# Autodesk Inventor assembly: RPI_2
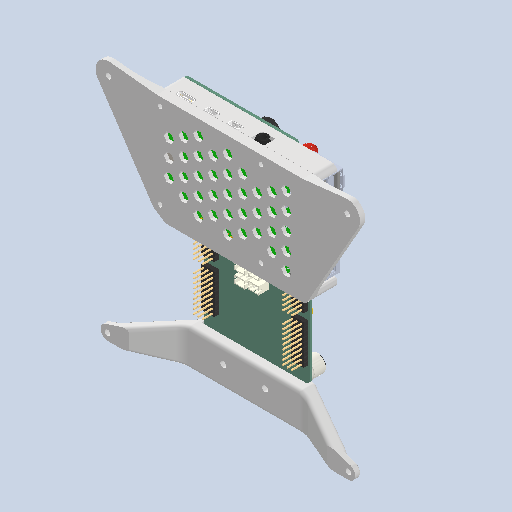
[picture p0: Inventor's stored thumbnail of the model, 512x512]
Saved by Autodesk Inventor 2023 (Build 270158000, 158)
## iProperties
Created: 2024-10-13
Part Number: RPI_2
Document SubType Name: Assembly
Designer: komputer
Author: komputer
## Documents named in this file (6)
- C:\Users\kamil\Documents\PROJECTS - repos\Robal-2.0\mechanics\RPI_2.iam
- C:\Users\kamil\Documents\PROJECTS - repos\Robal-2.0\mechanics\step\robal_rpi_ioBoard2\robal_rpi_ioBoard2.ipt
- C:\Users\kamil\Documents\PROJECTS - repos\Robal-2.0\mechanics\podstawa_rpi_1.ipt
- C:\Users\kamil\Documents\PROJECTS - repos\Robal-2.0\mechanics\podstawa_rpi_board_2.ipt
- C:\Users\kamil\Documents\PROJECTS - repos\Robal-2.0\mechanics\rpi_wspornik.ipt
- C:\Users\kamil\Documents\PROJECTS - repos\Robal-2.0\electronics\step\Raspberry Pi 4 Model B\Raspberry Pi 4 Model B.ipt
## Components (5 placed, 5 different names)
1. robal_rpi_ioBoard2:1 — Mate:1, Mate:2, Mate:3, Mate:7, Mate:8, Mate:9
2. podstawa_rpi_1:1 — Mate:10, Mate:11, Mate:12
3. podstawa_rpi_board_2:1 — Mate:7, Mate:8, Mate:9
4. rpi_wspornik:1 — Mate:1, Mate:2, Mate:3, Mate:4, Mate:5, Mate:6, Mate:11, Mate:12
5. Raspberry Pi 4 Model B:1 — Mate:4, Mate:5, Mate:6, Mate:10
## Relationships (12: Mate 12)
- Mate:1: robal_rpi_ioBoard2:1 ↔ rpi_wspornik:1
- Mate:2: robal_rpi_ioBoard2:1 ↔ rpi_wspornik:1
- Mate:3: robal_rpi_ioBoard2:1 ↔ rpi_wspornik:1
- Mate:4: rpi_wspornik:1 ↔ Raspberry Pi 4 Model B:1
- Mate:5: rpi_wspornik:1 ↔ Raspberry Pi 4 Model B:1
- Mate:6: rpi_wspornik:1 ↔ Raspberry Pi 4 Model B:1
- Mate:7: robal_rpi_ioBoard2:1 ↔ podstawa_rpi_board_2:1
- Mate:8: robal_rpi_ioBoard2:1 ↔ podstawa_rpi_board_2:1
- Mate:9: robal_rpi_ioBoard2:1 ↔ podstawa_rpi_board_2:1
- Mate:10: podstawa_rpi_1:1 ↔ Raspberry Pi 4 Model B:1
- Mate:11: podstawa_rpi_1:1 ↔ rpi_wspornik:1
- Mate:12: podstawa_rpi_1:1 ↔ rpi_wspornik:1
